# Autodesk Inventor assembly: joint1
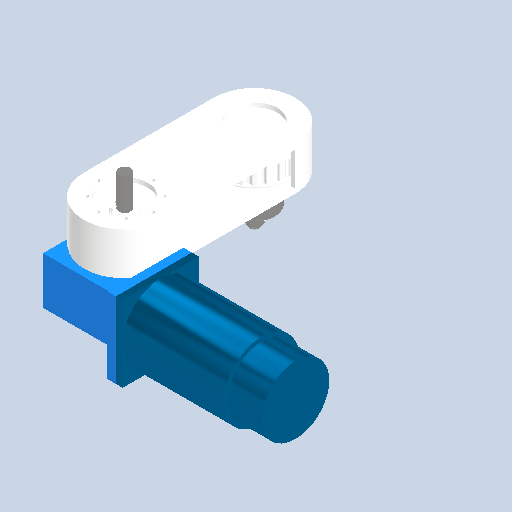
[picture p0: Inventor's stored thumbnail of the model, 512x512]
Saved by Autodesk Inventor 2025.3 (Build 293356030, 356C)
## iProperties
Created: 2025-09-07
Part Number: joint1
Document SubType Name: Assembly
Designer: MSI
Mass: 4008.4 g
Surface Area: 2679.28 cm^2
Volume: 2052.25 cm^3
Density: 1.95317 g/cm^3
Author: MSI
## Documents named in this file (7)
- C:\Users\MSI\Desktop\Project\11. 로봇팔\Robot Arm Model\Robot_Arm_6_v1\joint1.iam
- C:\Users\MSI\Desktop\Project\11. 로봇팔\Robot Arm Model\Robot_Arm_6_v1\joint1_frame.ipt
- C:\Users\MSI\Desktop\Project\11. 로봇팔\Robot Arm Model\Robot_Arm_6_v1\NMRV30_motor.iam
- C:\Users\MSI\Desktop\Project\11. 로봇팔\Robot Arm Model\Robot_Arm_6_v1\motor_shaft.ipt
- C:\Users\MSI\Desktop\Project\11. 로봇팔\Robot Arm Model\Robot_Arm_6_v1\belt_pulley_1.ipt
- C:\Users\MSI\Desktop\Project\11. 로봇팔\Robot Arm Model\Robot_Arm_6_v1\belt_pulley_2.ipt
- C:\Users\MSI\Desktop\Project\11. 로봇팔\Robot Arm Model\Robot_Arm_6_v1\encoder.ipt
## Components (6 placed, 6 different names)
1. joint1_frame:1 — 강체:1, 강체:2, 강체:4, 회전:1
2. NMRV30_motor:1 [sub-assembly] — 강체:3, 강체:4
3. motor_shaft:1 — 강체:3
4. 동기식 풀리1:1 — 강체:2
5. 동기식 풀리2:1 — 강체:1
6. encoder:1 — 회전:1
## Relationships (5: WeldJoint 4, RevoluteJoint 1)
- 강체:1 [WeldJoint] (-10 mm): joint1_frame:1 ↔ 동기식 풀리2:1
- 강체:2 [WeldJoint] (-7 mm): joint1_frame:1 ↔ 동기식 풀리1:1
- 강체:3 [WeldJoint]: NMRV30_motor:1 ↔ motor_shaft:1
- 강체:4 [WeldJoint]: joint1_frame:1 ↔ NMRV30_motor:1
- 회전:1 [RevoluteJoint]: joint1_frame:1 ↔ encoder:1
